# Autodesk Inventor assembly: Ring
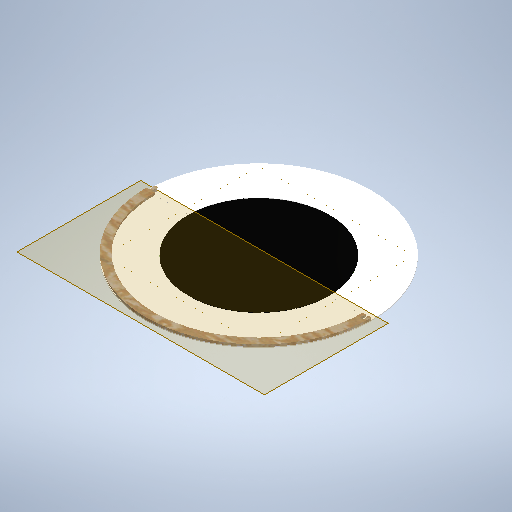
[picture p0: Inventor's stored thumbnail of the model, 512x512]
Saved by Autodesk Inventor 2025.2 (Build 292293000, 293)
## iProperties
Created: 2024-11-19
Part Number: Ring
Document SubType Name: Assembly
Designer: jaros
Author: jaros
## Documents named in this file (4)
- C:\Users\jaros\Downloads\Ring.iam
- C:\Users\jaros\Downloads\RingBlack.ipt
- C:\Users\jaros\Downloads\RingWhite.ipt
- C:\Users\jaros\Downloads\barrier.ipt
## Components (4 placed, 3 different names)
1. RingBlack:1 — Flush:1, Flush:2, Mate:2
2. RingWhite:1 — Flush:1, Flush:2, Flush:3, Mate:1, Flush:4, Flush:5
3. RingWhite:2 — Flush:3, Mate:1, Mate:2
4. barrier:1 — Flush:4, Flush:5
## Relationships (7: Flush 5, Mate 2)
- Flush:1: RingBlack:1 ↔ RingWhite:1
- Flush:2: RingBlack:1 ↔ RingWhite:1
- Flush:3: RingWhite:1 ↔ RingWhite:2
- Mate:1: RingWhite:1 ↔ RingWhite:2
- Mate:2: RingBlack:1 ↔ RingWhite:2
- Flush:4: RingWhite:1 ↔ barrier:1
- Flush:5: RingWhite:1 ↔ barrier:1
